# Autodesk Inventor assembly: Assemdrbly1dragon_assm
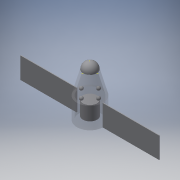
[picture p0: Inventor's stored thumbnail of the model, 180x180]
Saved by Autodesk Inventor 2018 (Build 220112000, 112)
## iProperties
Created: 2018-04-22
Part Number: Assemdrbly1dragon_assm
Document SubType Name: Assembly
Designer: atbin
Mass: 2.38285e+07 g
Surface Area: 1.5949e+06 cm^2
Volume: 2.58741e+07 cm^3
Density: 0.920941 g/cm^3
Author: atbin
## Documents named in this file (8)
- C:\Users\atbin\OneDrive\Documents\Stanford AA\SADC 279C\DragonCAD\Assemdrbly1dragon_assm.iam
- C:\Users\atbin\OneDrive\Documents\Stanford AA\SADC 279C\DragonCAD\pressurechamber.ipt
- C:\Users\atbin\OneDrive\Documents\Stanford AA\SADC 279C\DragonCAD\cargotrunk.ipt
- C:\Users\atbin\OneDrive\Documents\Stanford AA\SADC 279C\DragonCAD\nosecone.ipt
- C:\Users\atbin\OneDrive\Documents\Stanford AA\SADC 279C\DragonCAD\dracothruster.ipt
- C:\Users\atbin\OneDrive\Documents\Stanford AA\SADC 279C\DragonCAD\cargo.ipt
- C:\Users\atbin\OneDrive\Documents\Stanford AA\SADC 279C\DragonCAD\solarpanel.ipt
- C:\Users\atbin\OneDrive\Documents\Stanford AA\SADC 279C\DragonCAD\solarpanel_MIR.ipt
## Components (10 placed, 7 different names)
1. pressurechamber:1 — Mate:1, Mate:2, Mate:3, Mate:4, Tangent:1, Tangent:2, Mate:5
2. cargotrunk:1 — Mate:1, Mate:2, Flush:1, Mate:8, Flush:2
3. nosecone:1 — Mate:3, Mate:4, Mate:7
4. cargo:1 — Mate:7, Flush:1
5. solarpanel:1 — Flush:2, Flush:3, Mate:9
6. solarpanel_MIR:1 — Mate:10, Mate:11
7. dracothruster:1 — Tangent:1, Tangent:2, Mate:6
8. dracothruster:2
9. dracothruster:3
10. dracothruster:4
## Component patterns: (4 elements, first: dracothruster:1)
## Relationships (16: Mate 11, Flush 3, Tangent 2)
- Mate:1: pressurechamber:1 ↔ cargotrunk:1
- Mate:2: pressurechamber:1 ↔ cargotrunk:1
- Mate:3: pressurechamber:1 ↔ nosecone:1
- Mate:4: pressurechamber:1 ↔ nosecone:1
- Tangent:1: pressurechamber:1 ↔ dracothruster:1
- Tangent:2: pressurechamber:1 ↔ dracothruster:1
- Mate:5: pressurechamber:1
- Mate:6: dracothruster:1
- Mate:7: nosecone:1 ↔ cargo:1
- Flush:1 (500 mm): cargotrunk:1 ↔ cargo:1
- Mate:8: cargotrunk:1
- Flush:2: cargotrunk:1 ↔ solarpanel:1
- Flush:3 (1850 mm): solarpanel:1
- Mate:9 (-50 mm): solarpanel:1
- Mate:10 (-50 mm): solarpanel_MIR:1
- Mate:11 (1850 mm): solarpanel_MIR:1
